# Autodesk Inventor assembly: Locking
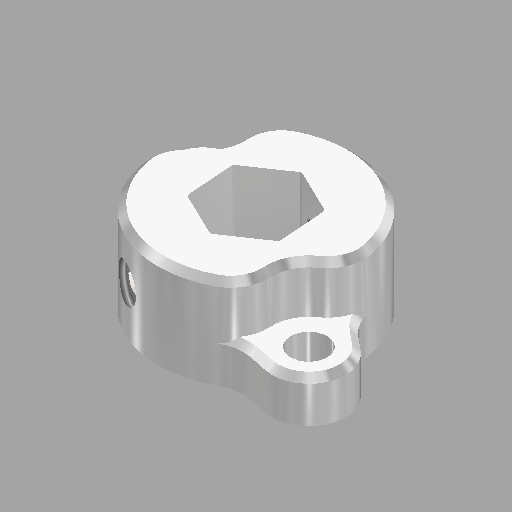
[picture p0: Inventor's stored thumbnail of the model, 512x512]
Saved by Autodesk Inventor 2027 (Build 310192060, 192F)
## iProperties
Created: 2026-06-26
Part Number: Locking
Document SubType Name: Assembly
Designer: opore
Author: opore
## Documents named in this file (3)
- H:\Autodesk\AirBrake\AirBrakeReal\Locking.iam
- H:\Autodesk\AirBrake\AirBrakeReal\ShaftHolder.ipt
- C:\Users\opore\OneDrive\Documents\Inventor\Content Center Files\R2027\en-US\AS 1421(2)\AS 1421 - M3 x 4 Cup Point.ipt
## Components (3 placed, 2 different names)
1. ShaftHolder:1
2. AS 1421 Cup Point - Metric M3 x 4 Cup Point:1
3. AS 1421 Cup Point - Metric M3 x 4 Cup Point:2
## Relationships (2: RevoluteJoint 2)
- [RevoluteJoint]: ShaftHolder:1 ↔ AS 1421 Cup Point - Metric M3 x 4 Cup Point:2
- [RevoluteJoint]: ShaftHolder:1 ↔ AS 1421 Cup Point - Metric M3 x 4 Cup Point:1
